# Autodesk Inventor assembly: aaa_001_ring
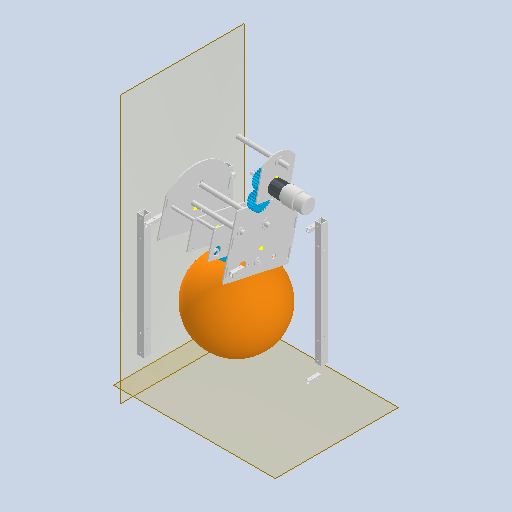
[picture p0: Inventor's stored thumbnail of the model, 512x512]
Saved by Autodesk Inventor 2025.2 (Build 292293000, 293)
## iProperties
Created: 2024-12-20
Part Number: aaa_001_ring
Document SubType Name: Assembly
Designer: yuki0520
Author: yuki0520
## Documents named in this file (6)
- C:\Users\haruy\Documents\ロボコン\NHK2025\cad\nagahisa\tanaka_dribll\2025_nhk\tanaka\drible\aaa_001_ring.iam
- C:\Users\haruy\Documents\ロボコン\NHK2025\cad\nagahisa\tanaka_dribll\2025_nhk\tanaka\nageru\smallring\small_kaku_2020_tka.ipt
- C:\Users\haruy\Documents\ロボコン\NHK2025\cad\nagahisa\tanaka_dribll\2025_nhk\tanaka\object\ball.ipt
- C:\Users\haruy\Documents\ロボコン\NHK2025\cad\nagahisa\tanaka_dribll\2025_nhk\tanaka\nageru\smallring\small_kaku_1010_bridge_1020.ipt
- C:\Users\haruy\Documents\ロボコン\NHK2025\cad\nagahisa\tanaka_dribll\2025_nhk\tanaka\nageru\smallring\small_kaku_1010_santen_1020.ipt
- C:\Users\haruy\Documents\ロボコン\NHK2025\cad\nagahisa\tanaka_dribll\2025_nhk\tanaka\drible\aaa_0011_wheel.iam
## Components (9 placed, 5 different names)
1. small_kaku_2020_tka:2 — メイト:1, 挿入:23, 挿入:43, 挿入:71
2. small_kaku_2020_tka:3 — 挿入:39, 挿入:40, 挿入:50, 挿入:67, 挿入:72
3. small_kaku_2020_tka:4 — 挿入:29, メイト:2, 挿入:54, 挿入:74
4. ball:1
5. small_kaku_1010_bridge_1020:1 — 挿入:23, 挿入:29, 挿入:43, 挿入:54, 挿入:70, 挿入:75
6. small_kaku_1010_santen_1020:1 — 挿入:40, 挿入:67
7. small_kaku_1010_santen_1020:2
8. small_kaku_1010_santen_1020:3 — 挿入:39, 挿入:50, 挿入:73
9. aaa_0011_wheel:1 [sub-assembly] — 挿入:70, 挿入:71, 挿入:72, 挿入:73, 挿入:74, 挿入:75
## Relationships (16: Insert 14, Mate 2)
- メイト:1 [Mate]: small_kaku_2020_tka:2
- 挿入:23 [Insert]: small_kaku_2020_tka:2 ↔ small_kaku_1010_bridge_1020:1
- 挿入:29 [Insert]: small_kaku_2020_tka:4 ↔ small_kaku_1010_bridge_1020:1
- メイト:2 [Mate]: small_kaku_2020_tka:4
- 挿入:39 [Insert]: small_kaku_2020_tka:3 ↔ small_kaku_1010_santen_1020:3
- 挿入:40 [Insert]: small_kaku_2020_tka:3 ↔ small_kaku_1010_santen_1020:1
- 挿入:43 [Insert]: small_kaku_2020_tka:2 ↔ small_kaku_1010_bridge_1020:1
- 挿入:50 [Insert]: small_kaku_2020_tka:3 ↔ small_kaku_1010_santen_1020:3
- 挿入:54 [Insert]: small_kaku_2020_tka:4 ↔ small_kaku_1010_bridge_1020:1
- 挿入:67 [Insert]: small_kaku_2020_tka:3 ↔ small_kaku_1010_santen_1020:1
- 挿入:70 [Insert]: small_kaku_1010_bridge_1020:1 ↔ aaa_0011_wheel:1
- 挿入:71 [Insert]: small_kaku_2020_tka:2 ↔ aaa_0011_wheel:1
- 挿入:72 [Insert]: small_kaku_2020_tka:3 ↔ aaa_0011_wheel:1
- 挿入:73 [Insert]: small_kaku_1010_santen_1020:3 ↔ aaa_0011_wheel:1
- 挿入:74 [Insert]: small_kaku_2020_tka:4 ↔ aaa_0011_wheel:1
- 挿入:75 [Insert]: small_kaku_1010_bridge_1020:1 ↔ aaa_0011_wheel:1
